# Autodesk Inventor assembly: Servo_Ku_asm
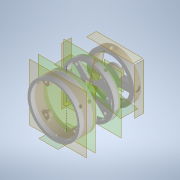
[picture p0: Inventor's stored thumbnail of the model, 180x180]
Saved by Autodesk Inventor 2020 (Build 240168000, 168)
## iProperties
Created: 2022-02-16
Part Number: Servo_Ku_asm
Document SubType Name: Assembly
Designer: sp
Author: sp
## Documents named in this file (4)
- C:\Users\sp\Documents\Rocket\rocket\CAD\Servo_Ku_asm.iam
- C:\Users\sp\Documents\Rocket\rocket\CAD\Servo_Kupplung.ipt
- C:\Users\sp\Documents\Rocket\rocket\CAD\Servo_holder.ipt
- C:\Users\sp\Documents\Rocket\rocket\CAD\Verbindungsring.ipt
## Components (3 placed, 3 different names)
1. Servo_Kupplung:1
2. Servo_holder:1 — Einfügen:2, Passend:1
3. Verbindungsring:1 — Einfügen:2, Passend:1
## Relationships (2: Insert 1, Mate 1)
- Einfügen:2 [Insert] (20 mm): Servo_holder:1 ↔ Verbindungsring:1
- Passend:1 [Mate]: Servo_holder:1 ↔ Verbindungsring:1
